# Autodesk Inventor assembly: Chassis, Wheels, and Drive Train Assembly
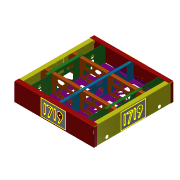
[picture p0: Inventor's stored thumbnail of the model, 180x180]
Saved by Autodesk Inventor 2015 (Build 190159000, 159)
## iProperties
Created: 2015-01-24
Part Number: Chassis, Wheels, and Drive Train Assembly
Document SubType Name: Assembly
Designer: Peter
Author: Peter
## Documents named in this file (3)
- T:\FILES\FIRST-Team-1719-CAD-Team\2015 Robot CAD\Chassis, Wheels, and Drive Train\Chassis, Wheels, and Drive Train Assembly.iam
- T:\FILES\FIRST-Team-1719-CAD-Team\2015 Robot CAD\Chassis, Wheels, and Drive Train\Chassis\Full chassis-3.iam
- T:\FILES\FIRST-Team-1719-CAD-Team\2015 Robot CAD\Number Plate\Number Plate.ipt
## Components (5 placed, 2 different names)
1. Full chassis-3:1 [sub-assembly] — Mate:1, Mate:2, Mate:3, Mate:4, Flush:1, Flush:2, Flush:3, Flush:4, Flush:5, Flush:6, Flush:7, Flush:8
2. Number Plate:1 — Mate:3, Flush:1, Flush:7
3. Number Plate:2 — Mate:4, Flush:2, Flush:6
4. Number Plate:3 — Mate:1, Flush:3, Flush:5
5. Number Plate:4 — Mate:2, Flush:4, Flush:8
## Relationships (12: Flush 8, Mate 4)
- Mate:1: Full chassis-3:1 ↔ Number Plate:3
- Mate:2: Full chassis-3:1 ↔ Number Plate:4
- Mate:3: Full chassis-3:1 ↔ Number Plate:1
- Mate:4: Full chassis-3:1 ↔ Number Plate:2
- Flush:1 (6.35 mm): Full chassis-3:1 ↔ Number Plate:1
- Flush:2 (6.35 mm): Full chassis-3:1 ↔ Number Plate:2
- Flush:3 (6.35 mm): Full chassis-3:1 ↔ Number Plate:3
- Flush:4 (6.35 mm): Full chassis-3:1 ↔ Number Plate:4
- Flush:5 (234.95 mm): Full chassis-3:1 ↔ Number Plate:3
- Flush:6 (234.95 mm): Full chassis-3:1 ↔ Number Plate:2
- Flush:7 (234.95 mm): Full chassis-3:1 ↔ Number Plate:1
- Flush:8 (234.95 mm): Full chassis-3:1 ↔ Number Plate:4
